# Autodesk Inventor assembly: Intake
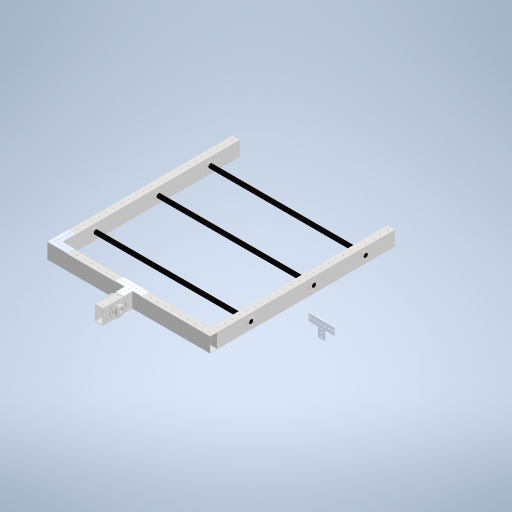
[picture p0: Inventor's stored thumbnail of the model, 512x512]
Saved by Autodesk Inventor 2023.2 (Build 272271000, 271)
## iProperties
Created: 2023-03-19
Part Number: Intake
Document SubType Name: Assembly
Designer: matth
Author: matth
## Documents named in this file (9)
- D:\CAD\2023 T3\Intake\Intake.iam
- D:\CAD\2023 T3\Intake\intake versa.ipt
- D:\CAD\2023 T3\Intake\Flanged Bearing.ipt
- D:\CAD\2023 T3\Intake\intake hex.ipt
- D:\CAD\2023 T3\Intake\intake base.ipt
- C:\Users\matth\Documents\GitHub\CAD\Stock\Versa System\Gussets\90 Degree Gusset.ipt
- C:\Users\matth\Documents\GitHub\CAD\Stock\Versa System\Gussets\Small T-VersaChassis Gusset.ipt
- D:\CAD\2023 T3\Intake\wrist attatchment.ipt
- D:\CAD\2023 T3\Intake\1_2” Hex Bore Aluminum VersaHub (217-2592).ipt
## Components (24 placed, 8 different names)
1. intake versa:1 — Insert:1, Insert:2, Insert:3, Insert:10, Insert:11, Insert:12
2. intake versa:2 — Insert:4, Insert:5, Insert:6, Insert:7, Insert:8, Insert:9, Mate:4, Mate:5
3. Flanged Bearing:1 — Insert:5
4. Flanged Bearing:2 — Insert:4
5. Flanged Bearing:3 — Insert:9, Insert:16
6. Flanged Bearing:4 — Insert:6
7. Flanged Bearing:5 — Insert:7, Insert:17
8. Flanged Bearing:6 — Insert:8
9. Flanged Bearing:7 — Insert:10
10. Flanged Bearing:8 — Insert:11
11. Flanged Bearing:9 — Insert:3, Insert:14
12. Flanged Bearing:10 — Insert:12
13. Flanged Bearing:11 — Insert:2, Insert:15
14. Flanged Bearing:12 — Insert:1, Insert:13
15. intake hex:1 — Insert:13, Insert:17
16. intake hex:2 — Insert:14
17. intake hex:3 — Insert:15, Insert:16
18. intake base:1 — Mate:1, Mate:2, Mate:3, Mate:8, Mate:9, Mate:10, Mate:11
19. 90 Degree Gusset:1 — Mate:1, Mate:2, Mate:3, Mate:4, Mate:5
20. Small T-VersaChassis Gusset:1 — Mate:9, Mate:10, Mate:11, Mate:12
21. Small T-VersaChassis Gusset:2
22. wrist attatchment:1 — Mate:8, Mate:12, Mate:13, Mate:14
23. 1_2” Hex Bore Aluminum VersaHub (217-2592):1 — Mate:13
24. 1_2” Hex Bore Aluminum VersaHub (217-2592):2 — Mate:14
## Relationships (29: Insert 17, Mate 12)
- Insert:1: intake versa:1 ↔ Flanged Bearing:12
- Insert:2: intake versa:1 ↔ Flanged Bearing:11
- Insert:3: intake versa:1 ↔ Flanged Bearing:9
- Insert:4: intake versa:2 ↔ Flanged Bearing:2
- Insert:5: intake versa:2 ↔ Flanged Bearing:1
- Insert:6: intake versa:2 ↔ Flanged Bearing:4
- Insert:7: intake versa:2 ↔ Flanged Bearing:5
- Insert:8: intake versa:2 ↔ Flanged Bearing:6
- Insert:9: intake versa:2 ↔ Flanged Bearing:3
- Insert:10: intake versa:1 ↔ Flanged Bearing:7
- Insert:11: intake versa:1 ↔ Flanged Bearing:8
- Insert:12: intake versa:1 ↔ Flanged Bearing:10
- Insert:13: Flanged Bearing:12 ↔ intake hex:1
- Insert:14: Flanged Bearing:9 ↔ intake hex:2
- Insert:15: Flanged Bearing:11 ↔ intake hex:3
- Insert:16: Flanged Bearing:3 ↔ intake hex:3
- Insert:17: Flanged Bearing:5 ↔ intake hex:1
- Mate:1: intake base:1 ↔ 90 Degree Gusset:1
- Mate:2: intake base:1 ↔ 90 Degree Gusset:1
- Mate:3: intake base:1 ↔ 90 Degree Gusset:1
- Mate:4: intake versa:2 ↔ 90 Degree Gusset:1
- Mate:5: intake versa:2 ↔ 90 Degree Gusset:1
- Mate:8: intake base:1 ↔ wrist attatchment:1
- Mate:9: intake base:1 ↔ Small T-VersaChassis Gusset:1
- Mate:10: intake base:1 ↔ Small T-VersaChassis Gusset:1
- Mate:11: intake base:1 ↔ Small T-VersaChassis Gusset:1
- Mate:12: Small T-VersaChassis Gusset:1 ↔ wrist attatchment:1
- Mate:13: wrist attatchment:1 ↔ 1_2” Hex Bore Aluminum VersaHub (217-2592):1
- Mate:14: wrist attatchment:1 ↔ 1_2” Hex Bore Aluminum VersaHub (217-2592):2
